# Autodesk Inventor assembly: 000-hand-grab-v5
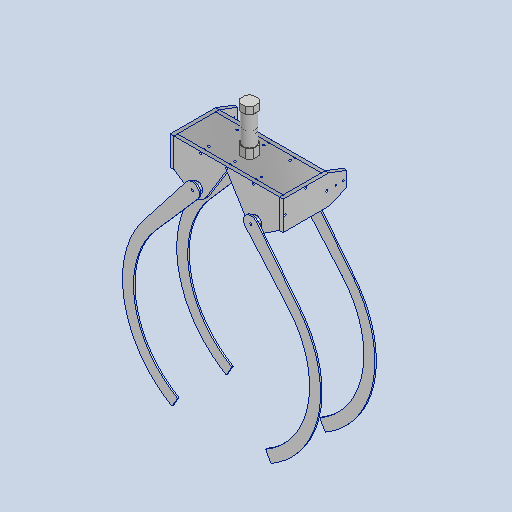
[picture p0: Inventor's stored thumbnail of the model, 512x512]
Saved by Autodesk Inventor 2025.2 (Build 292293000, 293)
## iProperties
Created: 2025-05-11
Part Number: 000-hand-grab-v5
Document SubType Name: Assembly
Designer: haruy
Author: haruy
## Documents named in this file (10)
- C:\Users\haruy\Documents\ロボコン\NHK2025\cad\nagahisa\hand\grab\000-hand-grab-v5.iam
- C:\Users\haruy\Documents\ロボコン\NHK2025\cad\nagahisa\hand\grab\hand-grab-v5-Plate-1.ipt
- C:\Users\haruy\Documents\ロボコン\NHK2025\cad\000_parts\エアシリンダー\airclinder\CDJ2B16-15Z-B(0_1_0).iam
- C:\Users\haruy\Documents\ロボコン\NHK2025\cad\nagahisa\hand\grab\hand-grab-v5-Plate-2.ipt
- C:\Users\haruy\Documents\ロボコン\NHK2025\cad\nagahisa\hand\grab\hand-grab-v5-Plate-3.ipt
- C:\Users\haruy\Documents\ロボコン\NHK2025\cad\000_parts\ベアリング\10\bear_10_15_sn.ipt
- C:\Users\haruy\Documents\ロボコン\NHK2025\cad\nagahisa\belt_liner\SCBRJ10-13.iam
- C:\Users\haruy\Documents\ロボコン\NHK2025\cad\nagahisa\hand\grab\hand-grab-v5-shaft-1.ipt
- C:\Users\haruy\Documents\ロボコン\NHK2025\cad\nagahisa\hand\grab\hand-grab-v5-Plate-4.ipt
- C:\Users\haruy\Documents\ロボコン\NHK2025\cad\nagahisa\hand\grab\hand-grab-v5-Plate-5.ipt
## Components (21 placed, 9 different names)
1. hand-grab-v5-Plate-1:1 — 挿入:1, 角度:1, メイト:1, フラッシュ:1, フラッシュ:2, フラッシュ:3, フラッシュ:4, メイト:2, フラッシュ:7, メイト:3, メイト:4, フラッシュ:10, 角度:2, 角度:3
2. CDJ2B16-15Z-B(0_1_0):1 [sub-assembly] — 挿入:1, 挿入:2
3. hand-grab-v5-Plate-2:1 — 挿入:2, 角度:1
4. hand-grab-v5-Plate-3:1 — メイト:1, フラッシュ:1, フラッシュ:2, 挿入:4, 挿入:6, 挿入:11, 挿入:12, フラッシュ:8, フラッシュ:9
5. hand-grab-v5-Plate-3:2 — フラッシュ:3, フラッシュ:4, メイト:2, 挿入:3, 挿入:5
6. bear_10_15_sn:1 — 挿入:4, 挿入:9
7. bear_10_15_sn:2 — 挿入:6, 挿入:10
8. bear_10_15_sn:3 — 挿入:5, 挿入:8
9. bear_10_15_sn:4 — 挿入:3, 挿入:7
10. SCBRJ10-13:1 [sub-assembly] — 挿入:7
11. SCBRJ10-13:2 [sub-assembly] — 挿入:8
12. SCBRJ10-13:3 [sub-assembly] — 挿入:9
13. SCBRJ10-13:4 [sub-assembly] — 挿入:10
14. hand-grab-v5-shaft-1:1 — 挿入:12, 挿入:15, 挿入:16
15. hand-grab-v5-shaft-1:2 — 挿入:11, 挿入:13, 挿入:14
16. hand-grab-v5-Plate-4:1 — 挿入:13, フラッシュ:5, 角度:2
17. hand-grab-v5-Plate-4:2 — 挿入:14, フラッシュ:5
18. hand-grab-v5-Plate-4:3 — 挿入:16, フラッシュ:6, 角度:3
19. hand-grab-v5-Plate-4:4 — 挿入:15, フラッシュ:6
20. hand-grab-v5-Plate-5:1 — フラッシュ:9, メイト:4, フラッシュ:10
21. hand-grab-v5-Plate-5:2 — フラッシュ:7, メイト:3, フラッシュ:8
## Relationships (33: Insert 16, Flush 10, Mate 4, Angle 3)
- 挿入:1 [Insert]: hand-grab-v5-Plate-1:1 ↔ CDJ2B16-15Z-B(0_1_0):1
- 挿入:2 [Insert] (5.5 mm): CDJ2B16-15Z-B(0_1_0):1 ↔ hand-grab-v5-Plate-2:1
- 角度:1 [Angle] (0 deg): hand-grab-v5-Plate-1:1 ↔ hand-grab-v5-Plate-2:1
- メイト:1 [Mate]: hand-grab-v5-Plate-1:1 ↔ hand-grab-v5-Plate-3:1
- フラッシュ:1 [Flush]: hand-grab-v5-Plate-1:1 ↔ hand-grab-v5-Plate-3:1
- フラッシュ:2 [Flush]: hand-grab-v5-Plate-1:1 ↔ hand-grab-v5-Plate-3:1
- フラッシュ:3 [Flush]: hand-grab-v5-Plate-1:1 ↔ hand-grab-v5-Plate-3:2
- フラッシュ:4 [Flush]: hand-grab-v5-Plate-1:1 ↔ hand-grab-v5-Plate-3:2
- メイト:2 [Mate]: hand-grab-v5-Plate-1:1 ↔ hand-grab-v5-Plate-3:2
- 挿入:3 [Insert]: hand-grab-v5-Plate-3:2 ↔ bear_10_15_sn:4
- 挿入:4 [Insert]: hand-grab-v5-Plate-3:1 ↔ bear_10_15_sn:1
- 挿入:5 [Insert]: hand-grab-v5-Plate-3:2 ↔ bear_10_15_sn:3
- 挿入:6 [Insert]: hand-grab-v5-Plate-3:1 ↔ bear_10_15_sn:2
- 挿入:7 [Insert]: bear_10_15_sn:4 ↔ SCBRJ10-13:1
- 挿入:8 [Insert]: bear_10_15_sn:3 ↔ SCBRJ10-13:2
- 挿入:9 [Insert]: bear_10_15_sn:1 ↔ SCBRJ10-13:3
- 挿入:10 [Insert]: bear_10_15_sn:2 ↔ SCBRJ10-13:4
- 挿入:11 [Insert] (-5 mm): hand-grab-v5-Plate-3:1 ↔ hand-grab-v5-shaft-1:2
- 挿入:12 [Insert] (-5 mm): hand-grab-v5-Plate-3:1 ↔ hand-grab-v5-shaft-1:1
- 挿入:13 [Insert]: hand-grab-v5-shaft-1:2 ↔ hand-grab-v5-Plate-4:1
- 挿入:14 [Insert]: hand-grab-v5-shaft-1:2 ↔ hand-grab-v5-Plate-4:2
- 挿入:15 [Insert]: hand-grab-v5-shaft-1:1 ↔ hand-grab-v5-Plate-4:4
- 挿入:16 [Insert]: hand-grab-v5-shaft-1:1 ↔ hand-grab-v5-Plate-4:3
- フラッシュ:5 [Flush]: hand-grab-v5-Plate-4:1 ↔ hand-grab-v5-Plate-4:2
- フラッシュ:6 [Flush]: hand-grab-v5-Plate-4:3 ↔ hand-grab-v5-Plate-4:4
- フラッシュ:7 [Flush]: hand-grab-v5-Plate-1:1 ↔ hand-grab-v5-Plate-5:2
- メイト:3 [Mate]: hand-grab-v5-Plate-1:1 ↔ hand-grab-v5-Plate-5:2
- フラッシュ:8 [Flush]: hand-grab-v5-Plate-3:1 ↔ hand-grab-v5-Plate-5:2
- フラッシュ:9 [Flush]: hand-grab-v5-Plate-3:1 ↔ hand-grab-v5-Plate-5:1
- メイト:4 [Mate]: hand-grab-v5-Plate-1:1 ↔ hand-grab-v5-Plate-5:1
- フラッシュ:10 [Flush]: hand-grab-v5-Plate-1:1 ↔ hand-grab-v5-Plate-5:1
- 角度:2 [Angle] (52 deg): hand-grab-v5-Plate-1:1 ↔ hand-grab-v5-Plate-4:1
- 角度:3 [Angle] (52 deg): hand-grab-v5-Plate-1:1 ↔ hand-grab-v5-Plate-4:3
